# Autodesk Inventor assembly: 5015 model
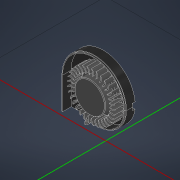
[picture p0: Inventor's stored thumbnail of the model, 180x180]
Saved by Autodesk Inventor 2022.2 (Build 262287010, 287A)
## iProperties
Created: 2022-03-16
Part Number: 5015 model
Document SubType Name: Assembly
Designer: sleib
Author: sleib
## Documents named in this file (3)
- C:\Users\sleib\Projekte\Voron-2\CAD\Inventor\Afterburner\Fan 5015 (stripped).iam
- C:\Users\sleib\Projekte\Voron-2\CAD\Inventor\Afterburner\Fan 5015 Turbine.ipt
- C:\Users\sleib\Projekte\Voron-2\CAD\Inventor\Afterburner\Fan 5015 Base.ipt
## Components (2 placed, 2 different names)
1. Fan 5015 Turbine:1 — Passend:1, Passend:2
2. Fan 5015 Base:1 — Passend:1, Passend:2, Fluchtend:1, Passend:3, Passend:4, Passend:5, Winkel:1
## Relationships (7: Mate 5, Flush 1, Angle 1)
- Passend:1 [Mate]: Fan 5015 Turbine:1 ↔ Fan 5015 Base:1
- Passend:2 [Mate] (1 mm): Fan 5015 Turbine:1 ↔ Fan 5015 Base:1
- Fluchtend:1 [Flush]: Fan 5015 Base:1
- Passend:3 [Mate]: Fan 5015 Base:1
- Passend:4 [Mate]: Fan 5015 Base:1
- Passend:5 [Mate]: Fan 5015 Base:1
- Winkel:1 [Angle] (0 deg): Fan 5015 Base:1
